# Autodesk Inventor assembly: Conveyer Belt Assembly
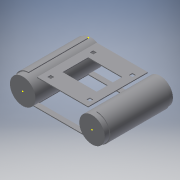
[picture p0: Inventor's stored thumbnail of the model, 180x180]
Saved by Autodesk Inventor 2019 (Build 230136000, 136)
## iProperties
Created: 2020-02-19
Part Number: Conveyer Belt Assembly
Document SubType Name: Assembly
Designer: JOHNWICK_58
Author: JOHNWICK_58
## Documents named in this file (3)
- C:\Users\LENOVO\Desktop\Abhishek\Conveyer Belt Assembly.iam
- C:\Users\LENOVO\Desktop\Abhishek\conveyer belt.ipt
- C:\Users\LENOVO\Desktop\Abhishek\Rollers for conveyer.ipt
## Components (3 placed, 2 different names)
1. Rollers for conveyer:1 — Mate:1
2. Rollers for conveyer:2 — Mate:2
3. conveyer belt:1 — Mate:1, Mate:2
## Relationships (2: Mate 2)
- Mate:1: Rollers for conveyer:1 ↔ conveyer belt:1
- Mate:2: Rollers for conveyer:2 ↔ conveyer belt:1
